# Autodesk Inventor assembly: back wheels
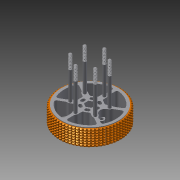
[picture p0: Inventor's stored thumbnail of the model, 180x180]
Saved by Autodesk Inventor 2014 SP1 (Build 180222100, 222)
## iProperties
Created: 2014-01-05
Part Number: back wheels
Document SubType Name: Assembly
Designer: Arpan
Author: Arpan
## Documents named in this file (4)
- C:\Users\Arpan\Documents\GitHub\2014buildCAD\chassisdrivetrain\chassis light\COTS items\back wheels.iam
- C:\Users\Arpan\Documents\GitHub\2014buildCAD\chassisdrivetrain\chassis light\COTS items\4 Perf ThruTread 500 Hex (1).ipt
- C:\Users\Arpan\Documents\GitHub\2014buildCAD\chassisdrivetrain\chassis light\COTS items\4 Inch Performance Wheel Tread.ipt
- C:\Users\Arpan\Documents\GitHub\2014buildCAD\chassisdrivetrain\chassis light\COTS items\91251A085.ipt
## Components (8 placed, 3 different names)
1. 4 Perf ThruTread 500 Hex (1):1 — Mate:1, Mate:2, Mate:3, Mate:4, Mate:5, Mate:6, Mate:7, Mate:8, Mate:9, Mate:10, Mate:11, Mate:12, Mate:13, Mate:14
2. 4 Inch Performance Wheel Tread:1 — Mate:1, Mate:2
3. 91251A085:1 — Mate:3, Mate:13
4. 91251A085:2 — Mate:4, Mate:14
5. 91251A085:3 — Mate:6, Mate:9
6. 91251A085:4 — Mate:5, Mate:10
7. 91251A085:5 — Mate:7, Mate:12
8. 91251A085:6 — Mate:8, Mate:11
## Relationships (14: Mate 14)
- Mate:1: 4 Perf ThruTread 500 Hex (1):1 ↔ 4 Inch Performance Wheel Tread:1
- Mate:2: 4 Perf ThruTread 500 Hex (1):1 ↔ 4 Inch Performance Wheel Tread:1
- Mate:3: 4 Perf ThruTread 500 Hex (1):1 ↔ 91251A085:1
- Mate:4: 4 Perf ThruTread 500 Hex (1):1 ↔ 91251A085:2
- Mate:5: 4 Perf ThruTread 500 Hex (1):1 ↔ 91251A085:4
- Mate:6: 4 Perf ThruTread 500 Hex (1):1 ↔ 91251A085:3
- Mate:7: 4 Perf ThruTread 500 Hex (1):1 ↔ 91251A085:5
- Mate:8: 4 Perf ThruTread 500 Hex (1):1 ↔ 91251A085:6
- Mate:9: 4 Perf ThruTread 500 Hex (1):1 ↔ 91251A085:3
- Mate:10: 4 Perf ThruTread 500 Hex (1):1 ↔ 91251A085:4
- Mate:11: 4 Perf ThruTread 500 Hex (1):1 ↔ 91251A085:6
- Mate:12: 4 Perf ThruTread 500 Hex (1):1 ↔ 91251A085:5
- Mate:13: 4 Perf ThruTread 500 Hex (1):1 ↔ 91251A085:1
- Mate:14: 4 Perf ThruTread 500 Hex (1):1 ↔ 91251A085:2
